# Autodesk Inventor assembly: pritlacne_kolecko_sestava
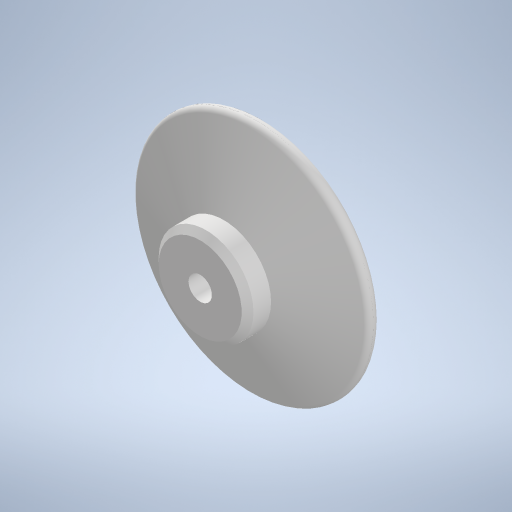
[picture p0: Inventor's stored thumbnail of the model, 512x512]
Saved by Autodesk Inventor 2023.1 (Build 271208000, 208)
## iProperties
Created: 2023-01-17
Part Number: pritlacne_kolecko_sestava
Document SubType Name: Assembly
Designer: zavrel
Author: zavrel
## Documents named in this file (2)
- C:\Users\zavrel\Documents\_OWNCLOUD_ACTUAL_WORK\GACR_Tensegrity\35_pohon_pro_Miletin\sestava_pohonu_SERVO\pritlacne_kolecko_sestava.iam
- C:\Users\zavrel\Documents\_OWNCLOUD_ACTUAL_WORK\GACR_Tensegrity\35_pohon_pro_Miletin\sestava_pohonu_SERVO\pritlacne_kolecko_polovina.ipt
## Components (2 placed, 1 different names)
1. pritlacne_kolecko_polovina:1 — Rigid:1
2. pritlacne_kolecko_polovina:2 — Rigid:1
## Relationships (1: WeldJoint 1)
- Rigid:1 [WeldJoint]: pritlacne_kolecko_polovina:1 ↔ pritlacne_kolecko_polovina:2
